# Autodesk Inventor assembly: electronics_perboard
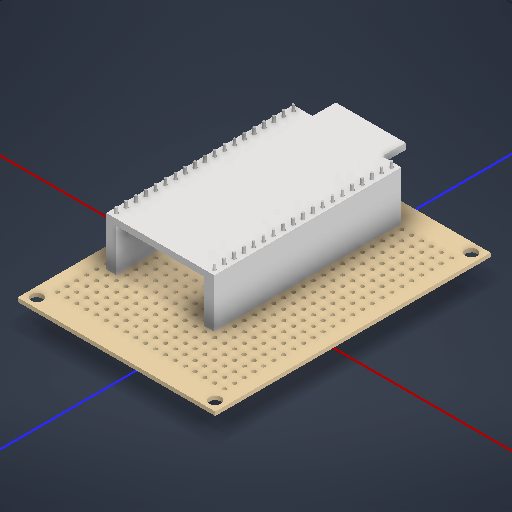
[picture p0: Inventor's stored thumbnail of the model, 512x512]
Saved by Autodesk Inventor 2025.2 (Build 292293000, 293)
## iProperties
Created: 2025-11-15
Part Number: electronics_perboard
Document SubType Name: Assembly
Designer: sam
Author: sam
## Documents named in this file (4)
- G:\projects\primary\auto-water-distribution-system\model\asm\module-command\electronics-command_perfboard.iam
- G:\projects\primary\auto-water-distribution-system\model\asm\general\perfboard-71x51x1.ipt
- G:\projects\primary\auto-water-distribution-system\model\asm\module-command\electronic-components\esp32-devkitc-v4.iam
- G:\projects\primary\auto-water-distribution-system\model\asm\general\pin-header-female.ipt
## Components (40 placed, 3 different names)
1. perfboard-71x51x1:1 — Mate:1, Mate:2, Mate:3
2. esp32-devkitc-v4:1 [sub-assembly] — Mate:4, Mate:5, Mate:6, Mate:7, Mate:8, Mate:9
3. pin-header-female:1 — Mate:2, Mate:3, Mate:5, Mate:6
4. pin-header-female:2
5. pin-header-female:3
6. pin-header-female:4
7. pin-header-female:5
8. pin-header-female:6
9. pin-header-female:7
10. pin-header-female:8
11. pin-header-female:9
12. pin-header-female:10
13. pin-header-female:11
14. pin-header-female:12
15. pin-header-female:13
16. pin-header-female:14
17. pin-header-female:15
18. pin-header-female:16
19. pin-header-female:17
20. pin-header-female:18
21. pin-header-female:19 — Mate:1, Mate:4
22. pin-header-female:20 — Mate:7, Mate:9
23. pin-header-female:21
24. pin-header-female:22
25. pin-header-female:23
26. pin-header-female:24
27. pin-header-female:25
28. pin-header-female:26
29. pin-header-female:27
30. pin-header-female:28
31. pin-header-female:29
32. pin-header-female:30
33. pin-header-female:31
34. pin-header-female:32
35. pin-header-female:33
36. pin-header-female:34
37. pin-header-female:35
38. pin-header-female:36
39. pin-header-female:37
40. pin-header-female:38 — Mate:8
## Component patterns: (19 elements, first: pin-header-female:1), (19 elements, first: pin-header-female:20)
## Relationships (9: Mate 9)
- Mate:1: perfboard-71x51x1:1 ↔ pin-header-female:19
- Mate:2: perfboard-71x51x1:1 ↔ pin-header-female:1
- Mate:3: perfboard-71x51x1:1 ↔ pin-header-female:1
- Mate:4: esp32-devkitc-v4:1 ↔ pin-header-female:19
- Mate:5: esp32-devkitc-v4:1 ↔ pin-header-female:1
- Mate:6: esp32-devkitc-v4:1 ↔ pin-header-female:1
- Mate:7: esp32-devkitc-v4:1 ↔ pin-header-female:20
- Mate:8: esp32-devkitc-v4:1 ↔ pin-header-female:38
- Mate:9: esp32-devkitc-v4:1 ↔ pin-header-female:20
